# Autodesk Inventor assembly: bellows_2
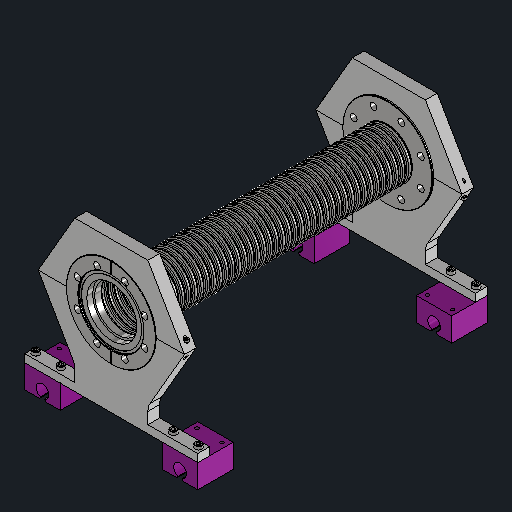
[picture p0: Inventor's stored thumbnail of the model, 512x512]
Saved by Autodesk Inventor 2027.1 (Build 311270010, 270A)
## iProperties
Created: 2026-06-24
Part Number: bellows_2
Document SubType Name: Assembly
Designer: shusu
Author: shusu
## Documents named in this file (3)
- C:\Users\queezz\Dropbox\Drawings\pihti-cad\bwllows-probe\bellows_2.iam
- C:\Users\queezz\Dropbox\Drawings\pihti-cad\bwllows-probe\bellows_bellows.ipt
- C:\Users\queezz\Dropbox\Drawings\pihti-cad\bwllows-probe\bellows_1.iam
## Components (3 placed, 2 different names)
1. bellows_bellows:1 — Insert:1, Insert:2
2. bellows_1:1 [sub-assembly] — Insert:2, Angle:1
3. bellows_1:2 [sub-assembly] — Insert:1, Angle:1
## Relationships (3: Insert 2, Angle 1)
- Insert:1 (-1 mm): bellows_bellows:1 ↔ bellows_1:2
- Insert:2 (1 mm): bellows_bellows:1 ↔ bellows_1:1
- Angle:1 (0 deg): bellows_1:1 ↔ bellows_1:2
